# Autodesk Inventor assembly: assembly
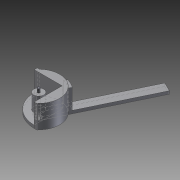
[picture p0: Inventor's stored thumbnail of the model, 180x180]
Saved by Autodesk Inventor 2012 (Build 160160000, 160)
## iProperties
Created: 2014-03-21
Part Number: assembly
Document SubType Name: Assembly
Designer: joe_000
Author: joe_000
## Documents named in this file (4)
- C:\dev\camera-multitouch\mounting-bracket\assembly.iam
- C:\dev\camera-multitouch\mounting-bracket\tv-mount.ipt
- C:\dev\camera-multitouch\mounting-bracket\arm.ipt
- C:\Users\joe_000\Documents\Inventor\Content Center Files\R2012\en-US\ANSI B18.6.7M(01)\ANSI B18.6.7M - M2.5x0.45 x 25(5).ipt
## Components (3 placed, 3 different names)
1. tv-mount:1 — Insert:1
2. arm:1 — Insert:1, Insert:2
3. Cross Recessed Pan Head Machine Screw - Type IA - Metric M2.5x0.45 x 25:1 — Insert:2
## Relationships (2: Insert 2)
- Insert:1: tv-mount:1 ↔ arm:1
- Insert:2: arm:1 ↔ Cross Recessed Pan Head Machine Screw - Type IA - Metric M2.5x0.45 x 25:1
